# Autodesk Inventor assembly: Support A Assembly Single LEFT
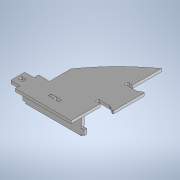
[picture p0: Inventor's stored thumbnail of the model, 180x180]
Saved by Autodesk Inventor 2020 (Build 240168000, 168)
## iProperties
Created: 2020-05-11
Part Number: Support A Assembly Single LEFT
Document SubType Name: Assembly
Designer: Dan Wikman
Author: Dan Wikman
## Documents named in this file (3)
- C:\Users\Dan Wikman\OneDrive\University Life\2020, Semester 1\METR4900 Honours Thesis\Full Scale Design\Support A Assembly Single LEFT.iam
- C:\Users\Dan Wikman\OneDrive\University Life\2020, Semester 1\METR4900 Honours Thesis\Full Scale Design\Layer 1 Plank.ipt
- C:\Users\Dan Wikman\OneDrive\University Life\2020, Semester 1\METR4900 Honours Thesis\Full Scale Design\Support A.ipt
## Components (2 placed, 2 different names)
1. Layer 1 Plank:1 — Flush:1, Mate:1, Mate:2
2. Support A:1 — Flush:1, Mate:1, Mate:2
## Relationships (3: Mate 2, Flush 1)
- Flush:1: Layer 1 Plank:1 ↔ Support A:1
- Mate:1 (0.5 mm): Layer 1 Plank:1 ↔ Support A:1
- Mate:2: Layer 1 Plank:1 ↔ Support A:1
